# Autodesk Inventor assembly: Gameboy NG
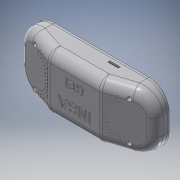
[picture p0: Inventor's stored thumbnail of the model, 180x180]
Saved by Autodesk Inventor 2016 SP1 (Build 200210100, 210)
## iProperties
Created: 2018-06-05
Part Number: Gameboy NG
Material: Générique
Document SubType Name: Assembly
Designer: dimercur
Author: dimercur
## Documents named in this file (13)
- D:\Users\dimercur\Documents\git\arm-ada-ng\hardware\Box\Gameboy NG.iam
- D:\Users\dimercur\Documents\git\arm-ada-ng\hardware\Box\STM32F746G-Disco.ipt
- D:\Users\dimercur\Documents\git\arm-ada-ng\hardware\Box\Partie Haute.ipt
- D:\Users\dimercur\Documents\Inventor\Content Center Files\R2016\fr-FR\BS 4183(4)\BS 4183 - M3 x 5(1) III.ipt
- D:\Users\dimercur\Documents\git\arm-ada-ng\hardware\Box\Button.ipt
- D:\Users\dimercur\Documents\git\arm-ada-ng\hardware\Box\Cross.ipt
- D:\Users\dimercur\Documents\git\arm-ada-ng\hardware\Box\Partie basse.ipt
- D:\Users\dimercur\Documents\Inventor\Content Center Files\R2016\fr-FR\ISO 7380-1\ISO 7380-1 - M3 x 6.ipt
- D:\Users\dimercur\Documents\git\arm-ada-ng\hardware\Box\Satellite Gauche.iam
- D:\Users\dimercur\Documents\Inventor\Content Center Files\R2016\fr-FR\NF E 25-111\NF E 25-111 - M2.5x6 Classe de qualité 4.8.ipt
- D:\Users\dimercur\Documents\git\arm-ada-ng\hardware\Box\Satellite Droit.iam
- D:\Users\dimercur\Documents\git\arm-ada-ng\hardware\Box\X-Nucleo-IKS01A1.ipt
- D:\Users\dimercur\Documents\git\arm-ada-ng\hardware\Box\PCB Wifi.ipt
## Components (26 placed, 12 different names)
1. STM32F746G-Disco:1 — Placage:1, Placage:2, Placage:3, Logement:1, Logement:2, Logement:3, Logement:4, Placage:27, Placage:28, Placage:29
2. Partie Haute:1 — Placage:1, Placage:2, Placage:3, Affleurement:1, Placage:4, Placage:6, Placage:8, Placage:9, Placage:10, Placage:11, Placage:12, Placage:13, Placage:14, Placage:15, Placage:16, Placage:17, Placage:18, Placage:19, Placage:20, Placage:21, Placage:22, Placage:23, Placage:24, Placage:25, Placage:26
3. BS 4183 Spécifications des vis et des écrous mécaniques - Série métrique - Métrique M3 x 5:1 — Logement:1
4. BS 4183 Spécifications des vis et des écrous mécaniques - Série métrique - Métrique M3 x 5:2 — Logement:2
5. BS 4183 Spécifications des vis et des écrous mécaniques - Série métrique - Métrique M3 x 5:3 — Logement:3
6. BS 4183 Spécifications des vis et des écrous mécaniques - Série métrique - Métrique M3 x 5:4 — Logement:4
7. Button:1 — Placage:9, Placage:14
8. Button:2 — Placage:6, Placage:10
9. Button:3 — Placage:11, Placage:13
10. Button:4 — Placage:8, Placage:12
11. Cross:1 — Placage:15, Placage:16, Placage:17
12. Dessous:1 — Placage:18, Placage:19, Placage:20, Logement:5, Logement:6, Logement:7, Logement:8
13. ISO 7380-1 M3 x 6:1 — Logement:5
14. ISO 7380-1 M3 x 6:2 — Logement:6
15. ISO 7380-1 M3 x 6:3 — Logement:7
16. ISO 7380-1 M3 x 6:4 — Logement:8
17. Satellite Gauche:1 [sub-assembly] — Placage:21, Placage:22, Placage:23, Logement:9, Logement:10, Logement:11
18. NF E 25-111 M2.5x6 Classe de qualité 4.8:1 — Logement:9
19. NF E 25-111 M2.5x6 Classe de qualité 4.8:2 — Logement:10
20. NF E 25-111 M2.5x6 Classe de qualité 4.8:3 — Logement:11
21. Satellite Droit:1 [sub-assembly] — Placage:24, Placage:25, Placage:26, Logement:12, Logement:13, Logement:14
22. NF E 25-111 M2.5x6 Classe de qualité 4.8:4 — Logement:12
23. NF E 25-111 M2.5x6 Classe de qualité 4.8:5 — Logement:13
24. NF E 25-111 M2.5x6 Classe de qualité 4.8:6 — Logement:14
25. X-Nucleo-IKS01A1:1 — Placage:30, Placage:31, Placage:32
26. PCB Wifi:1 — Placage:27, Placage:28, Placage:29, Placage:30, Placage:31, Placage:32
## Relationships (45: Mate 30, Insert 14, Flush 1)
- Placage:1 [Mate]: STM32F746G-Disco:1 ↔ Partie Haute:1
- Placage:2 [Mate]: STM32F746G-Disco:1 ↔ Partie Haute:1
- Placage:3 [Mate]: STM32F746G-Disco:1 ↔ Partie Haute:1
- Affleurement:1 [Flush]: Partie Haute:1
- Placage:4 [Mate]: Partie Haute:1
- Logement:1 [Insert]: STM32F746G-Disco:1 ↔ BS 4183 Spécifications des vis et des écrous mécaniques - Série métrique - Métrique M3 x 5:1
- Logement:2 [Insert]: STM32F746G-Disco:1 ↔ BS 4183 Spécifications des vis et des écrous mécaniques - Série métrique - Métrique M3 x 5:2
- Logement:3 [Insert]: STM32F746G-Disco:1 ↔ BS 4183 Spécifications des vis et des écrous mécaniques - Série métrique - Métrique M3 x 5:3
- Logement:4 [Insert]: STM32F746G-Disco:1 ↔ BS 4183 Spécifications des vis et des écrous mécaniques - Série métrique - Métrique M3 x 5:4
- Placage:6 [Mate]: Partie Haute:1 ↔ Button:2
- Placage:8 [Mate]: Partie Haute:1 ↔ Button:4
- Placage:9 [Mate]: Partie Haute:1 ↔ Button:1
- Placage:10 [Mate]: Partie Haute:1 ↔ Button:2
- Placage:11 [Mate]: Partie Haute:1 ↔ Button:3
- Placage:12 [Mate]: Partie Haute:1 ↔ Button:4
- Placage:13 [Mate]: Partie Haute:1 ↔ Button:3
- Placage:14 [Mate]: Partie Haute:1 ↔ Button:1
- Placage:15 [Mate]: Partie Haute:1 ↔ Cross:1
- Placage:16 [Mate] (0.5 mm): Partie Haute:1 ↔ Cross:1
- Placage:17 [Mate] (0.5 mm): Partie Haute:1 ↔ Cross:1
- Placage:18 [Mate]: Partie Haute:1 ↔ Dessous:1
- Placage:19 [Mate]: Partie Haute:1 ↔ Dessous:1
- Placage:20 [Mate]: Partie Haute:1 ↔ Dessous:1
- Logement:5 [Insert]: Dessous:1 ↔ ISO 7380-1 M3 x 6:1
- Logement:6 [Insert]: Dessous:1 ↔ ISO 7380-1 M3 x 6:2
- Logement:7 [Insert]: Dessous:1 ↔ ISO 7380-1 M3 x 6:3
- Logement:8 [Insert]: Dessous:1 ↔ ISO 7380-1 M3 x 6:4
- Placage:21 [Mate]: Partie Haute:1 ↔ Satellite Gauche:1
- Placage:22 [Mate]: Partie Haute:1 ↔ Satellite Gauche:1
- Placage:23 [Mate]: Partie Haute:1 ↔ Satellite Gauche:1
- Logement:9 [Insert]: Satellite Gauche:1 ↔ NF E 25-111 M2.5x6 Classe de qualité 4.8:1
- Logement:10 [Insert]: Satellite Gauche:1 ↔ NF E 25-111 M2.5x6 Classe de qualité 4.8:2
- Logement:11 [Insert]: Satellite Gauche:1 ↔ NF E 25-111 M2.5x6 Classe de qualité 4.8:3
- Placage:24 [Mate]: Partie Haute:1 ↔ Satellite Droit:1
- Placage:25 [Mate]: Partie Haute:1 ↔ Satellite Droit:1
- Placage:26 [Mate]: Partie Haute:1 ↔ Satellite Droit:1
- Logement:12 [Insert]: Satellite Droit:1 ↔ NF E 25-111 M2.5x6 Classe de qualité 4.8:4
- Logement:13 [Insert]: Satellite Droit:1 ↔ NF E 25-111 M2.5x6 Classe de qualité 4.8:5
- Logement:14 [Insert]: Satellite Droit:1 ↔ NF E 25-111 M2.5x6 Classe de qualité 4.8:6
- Placage:27 [Mate]: STM32F746G-Disco:1 ↔ PCB Wifi:1
- Placage:28 [Mate]: STM32F746G-Disco:1 ↔ PCB Wifi:1
- Placage:29 [Mate]: STM32F746G-Disco:1 ↔ PCB Wifi:1
- Placage:30 [Mate]: X-Nucleo-IKS01A1:1 ↔ PCB Wifi:1
- Placage:31 [Mate]: X-Nucleo-IKS01A1:1 ↔ PCB Wifi:1
- Placage:32 [Mate]: X-Nucleo-IKS01A1:1 ↔ PCB Wifi:1
